# Autodesk Inventor assembly: room1113
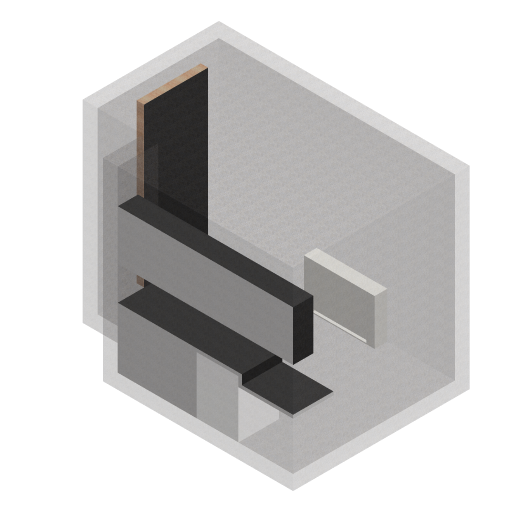
[picture p0: Inventor's stored thumbnail of the model, 512x512]
Saved by Autodesk Inventor 2023 (Build 270158000, 158)
## iProperties
Created: 2023-11-13
Part Number: room1113
Document SubType Name: Assembly
Designer: byfbi
Author: byfbi
## Documents named in this file (14)
- D:\INVENTOR\new kitchen\room1113.iam
- D:\INVENTOR\new kitchen\heater.ipt
- D:\INVENTOR\new kitchen\storage.ipt
- D:\INVENTOR\new kitchen\fridge.ipt
- D:\INVENTOR\new kitchen\small cupboard.ipt
- D:\INVENTOR\new kitchen\shelf.ipt
- D:\INVENTOR\new kitchen\room.ipt
- D:\INVENTOR\new kitchen\door.ipt
- D:\INVENTOR\new kitchen\air.ipt
- D:\INVENTOR\new kitchen\cupboard.ipt
- D:\INVENTOR\new kitchen\heating element.ipt
- D:\INVENTOR\new kitchen\new heating elements.ipt
- D:\INVENTOR\new kitchen\plane.ipt
- D:\INVENTOR\new kitchen\sensor.ipt
## Components (25 placed, 13 different names)
1. heater:1 — 表面齐平:1, 表面齐平:2, 表面齐平:3, 表面齐平:14, 表面齐平:15, 表面齐平:16, 配合:6, 配合:7, 配合:8
2. storage:1 — 表面齐平:4, 表面齐平:5, 表面齐平:6, 表面齐平:25, 表面齐平:26, 配合:9, 表面齐平:27, 表面齐平:28, 配合:10, 表面齐平:29, 表面齐平:30, 配合:11, 配合:12, 配合:13, 表面齐平:31, 配合:14, 配合:15, 表面齐平:32, 配合:16, 配合:17, 表面齐平:33, 配合:18, 配合:19, 表面齐平:34, 配合:20, 配合:21, 表面齐平:35, 配合:22, 配合:23, 表面齐平:36
3. fridge:1 — 配合:1, 表面齐平:7, 表面齐平:8, 配合:3
4. small cupboard:1 — 配合:1, 表面齐平:7, 表面齐平:8, 配合:2, 表面齐平:9, 表面齐平:11, 表面齐平:12, 表面齐平:23, 表面齐平:24
5. shelf:1 — 配合:2, 配合:3, 表面齐平:9, 表面齐平:10, 表面齐平:22
6. room:1 — 表面齐平:10, 表面齐平:11, 表面齐平:12, 表面齐平:13, 表面齐平:14, 表面齐平:16, 表面齐平:17, 配合:4, 表面齐平:18, 表面齐平:19, 表面齐平:20, 表面齐平:21, 表面齐平:37, 表面齐平:39, 表面齐平:40, 配合:24, 表面齐平:41, 表面齐平:43, 表面齐平:44, 表面齐平:45, 表面齐平:46, 表面齐平:47, 表面齐平:48, 表面齐平:49, 表面齐平:50, 表面齐平:51, 配合:25, 配合:26, 配合:27, 表面齐平:52, 表面齐平:53
7. door:1 — 表面齐平:17, 配合:4, 表面齐平:18
8. air:1 — 表面齐平:19, 表面齐平:20, 表面齐平:21
9. cupboard:1 — 配合:5, 表面齐平:23, 表面齐平:24
10. heating element:1 — 配合:6, 配合:7, 配合:8
11. new heating elements:1 — 表面齐平:29, 表面齐平:30, 配合:11
12. new heating elements:2 — 表面齐平:25, 表面齐平:26, 配合:9
13. new heating elements:3 — 表面齐平:27, 表面齐平:28, 配合:10
14. new heating elements:4 — 配合:12, 配合:13, 表面齐平:31
15. new heating elements:5 — 配合:14, 配合:15, 表面齐平:32
16. new heating elements:6 — 配合:16, 配合:17, 表面齐平:33
17. new heating elements:7 — 配合:18, 配合:19, 表面齐平:34
18. new heating elements:8 — 配合:20, 配合:21, 表面齐平:35
19. new heating elements:9 — 配合:22, 配合:23, 表面齐平:36
20. plane:1 — 表面齐平:39, 表面齐平:40, 配合:24
21. sensor:1 — 表面齐平:41, 表面齐平:43, 表面齐平:53
22. sensor:2 — 表面齐平:44, 表面齐平:45, 表面齐平:46
23. sensor:3 — 表面齐平:47, 表面齐平:48, 表面齐平:49
24. sensor:4 — 表面齐平:50, 表面齐平:51, 配合:25
25. sensor:5 — 配合:26, 配合:27, 表面齐平:52
## Relationships (78: Flush 51, Mate 27)
- 表面齐平:1 [Flush] (-150 mm): heater:1
- 表面齐平:2 [Flush] (-175 mm): heater:1
- 表面齐平:3 [Flush] (-45 mm): heater:1
- 表面齐平:4 [Flush]: storage:1
- 表面齐平:5 [Flush]: storage:1
- 表面齐平:6 [Flush]: storage:1
- 配合:1 [Mate]: fridge:1 ↔ small cupboard:1
- 表面齐平:7 [Flush]: fridge:1 ↔ small cupboard:1
- 表面齐平:8 [Flush]: fridge:1 ↔ small cupboard:1
- 配合:2 [Mate]: small cupboard:1 ↔ shelf:1
- 配合:3 [Mate]: fridge:1 ↔ shelf:1
- 表面齐平:9 [Flush]: small cupboard:1 ↔ shelf:1
- 表面齐平:10 [Flush]: shelf:1 ↔ room:1
- 表面齐平:11 [Flush]: small cupboard:1 ↔ room:1
- 表面齐平:12 [Flush]: small cupboard:1 ↔ room:1
- 表面齐平:13 [Flush] (-1000 mm): room:1
- 表面齐平:14 [Flush]: heater:1 ↔ room:1
- 表面齐平:15 [Flush]: heater:1
- 表面齐平:16 [Flush]: heater:1 ↔ room:1
- 表面齐平:17 [Flush]: room:1 ↔ door:1
- 配合:4 [Mate]: room:1 ↔ door:1
- 表面齐平:18 [Flush]: room:1 ↔ door:1
- 表面齐平:19 [Flush]: room:1 ↔ air:1
- 表面齐平:20 [Flush]: room:1 ↔ air:1
- 表面齐平:21 [Flush]: room:1 ↔ air:1
- 表面齐平:22 [Flush] (500 mm): shelf:1
- 配合:5 [Mate]: cupboard:1
- 表面齐平:23 [Flush]: small cupboard:1 ↔ cupboard:1
- 表面齐平:24 [Flush]: small cupboard:1 ↔ cupboard:1
- 配合:6 [Mate]: heater:1 ↔ heating element:1
- 配合:7 [Mate]: heater:1 ↔ heating element:1
- 配合:8 [Mate]: heater:1 ↔ heating element:1
- 表面齐平:25 [Flush]: storage:1 ↔ new heating elements:2
- 表面齐平:26 [Flush]: storage:1 ↔ new heating elements:2
- 配合:9 [Mate]: storage:1 ↔ new heating elements:2
- 表面齐平:27 [Flush]: storage:1 ↔ new heating elements:3
- 表面齐平:28 [Flush]: storage:1 ↔ new heating elements:3
- 配合:10 [Mate]: storage:1 ↔ new heating elements:3
- 表面齐平:29 [Flush]: storage:1 ↔ new heating elements:1
- 表面齐平:30 [Flush]: storage:1 ↔ new heating elements:1
- 配合:11 [Mate]: storage:1 ↔ new heating elements:1
- 配合:12 [Mate]: storage:1 ↔ new heating elements:4
- 配合:13 [Mate]: storage:1 ↔ new heating elements:4
- 表面齐平:31 [Flush]: storage:1 ↔ new heating elements:4
- 配合:14 [Mate]: storage:1 ↔ new heating elements:5
- 配合:15 [Mate]: storage:1 ↔ new heating elements:5
- 表面齐平:32 [Flush]: storage:1 ↔ new heating elements:5
- 配合:16 [Mate]: storage:1 ↔ new heating elements:6
- 配合:17 [Mate]: storage:1 ↔ new heating elements:6
- 表面齐平:33 [Flush]: storage:1 ↔ new heating elements:6
- 配合:18 [Mate]: storage:1 ↔ new heating elements:7
- 配合:19 [Mate]: storage:1 ↔ new heating elements:7
- 表面齐平:34 [Flush]: storage:1 ↔ new heating elements:7
- 配合:20 [Mate]: storage:1 ↔ new heating elements:8
- 配合:21 [Mate]: storage:1 ↔ new heating elements:8
- 表面齐平:35 [Flush]: storage:1 ↔ new heating elements:8
- 配合:22 [Mate]: storage:1 ↔ new heating elements:9
- 配合:23 [Mate]: storage:1 ↔ new heating elements:9
- 表面齐平:36 [Flush]: storage:1 ↔ new heating elements:9
- 表面齐平:37 [Flush] (-1610 mm): room:1
- 表面齐平:39 [Flush]: room:1 ↔ plane:1
- 表面齐平:40 [Flush]: room:1 ↔ plane:1
- 配合:24 [Mate]: room:1 ↔ plane:1
- 表面齐平:41 [Flush]: room:1 ↔ sensor:1
- 表面齐平:43 [Flush]: room:1 ↔ sensor:1
- 表面齐平:44 [Flush]: room:1 ↔ sensor:2
- 表面齐平:45 [Flush]: room:1 ↔ sensor:2
- 表面齐平:46 [Flush]: room:1 ↔ sensor:2
- 表面齐平:47 [Flush]: room:1 ↔ sensor:3
- 表面齐平:48 [Flush]: room:1 ↔ sensor:3
- 表面齐平:49 [Flush]: room:1 ↔ sensor:3
- 表面齐平:50 [Flush]: room:1 ↔ sensor:4
- 表面齐平:51 [Flush]: room:1 ↔ sensor:4
- 配合:25 [Mate]: room:1 ↔ sensor:4
- 配合:26 [Mate]: room:1 ↔ sensor:5
- 配合:27 [Mate]: room:1 ↔ sensor:5
- 表面齐平:52 [Flush]: room:1 ↔ sensor:5
- 表面齐平:53 [Flush]: room:1 ↔ sensor:1
